# Autodesk Inventor assembly: Encoder
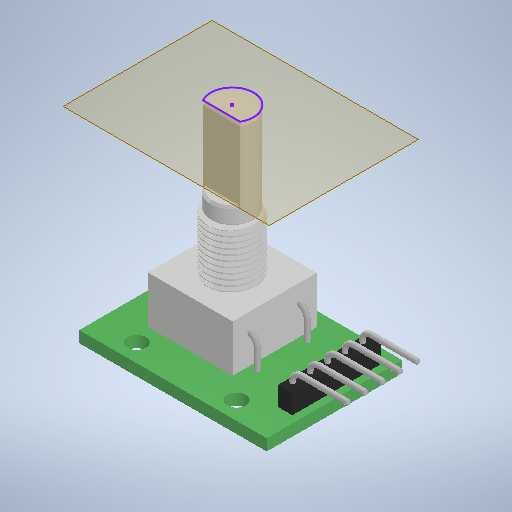
[picture p0: Inventor's stored thumbnail of the model, 512x512]
Saved by Autodesk Inventor 2025 (Build 290162000, 162)
## iProperties
Created: 2024-05-30
Part Number: Encoder
Document SubType Name: Assembly
Designer: AdminForWorker
Title: Encoder v1
Author: AdminForWorker
## Documents named in this file (9)
- C:\Users\hifzh\final_year\Design\TA-Design\part\sensors\Encoder v1\Encoder.iam
- C:\Users\hifzh\final_year\Design\TA-Design\part\sensors\Encoder v1\Component1.ipt
- C:\Users\hifzh\final_year\Design\TA-Design\part\sensors\Encoder v1\Component2.ipt
- C:\Users\hifzh\final_year\Design\TA-Design\part\sensors\Encoder v1\Component3.ipt
- C:\Users\hifzh\final_year\Design\TA-Design\part\sensors\Encoder v1\Component4.ipt
- C:\Users\hifzh\final_year\Design\TA-Design\part\sensors\Encoder v1\Component5.ipt
- C:\Users\hifzh\final_year\Design\TA-Design\part\sensors\Encoder v1\Component6.ipt
- C:\Users\hifzh\final_year\Design\TA-Design\part\sensors\Encoder v1\Component7.ipt
- C:\Users\hifzh\final_year\Design\TA-Design\part\sensors\Encoder v1\Part16.ipt
## Components (8 placed, 8 different names)
1. Component1:1 — Flush:1
2. Component2:1
3. Component3:1
4. Component4:1
5. Component5:1
6. Component6:1
7. Component7:1
8. Part16
## Relationships (1: Flush 1)
- Flush:1 (28.575 mm): Component1:1
